# Autodesk Inventor assembly: upper_body
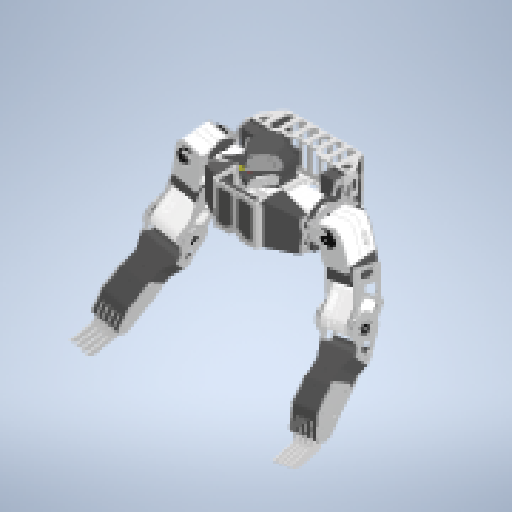
[picture p0: Inventor's stored thumbnail of the model, 512x512]
Saved by Autodesk Inventor 2024.1 (Build 281209000, 209)
## iProperties
Created: 2024-02-14
Part Number: upper_body
Document SubType Name: Assembly
Designer: hibik
Author: hibik
## Documents named in this file (3)
- C:\Users\hibik\Desktop\ロボメカ\HR\2024.02.11 Rl\02.11 ProtType\upper_body.iam
- C:\Users\hibik\Desktop\ロボメカ\HR\2024.02.11 Rl\02.11 ProtType\chest.iam
- C:\Users\hibik\Desktop\ロボメカ\HR\2024.02.11 Rl\02.11 ProtType\arm.iam
## Components (3 placed, 2 different names)
1. chest:1 [sub-assembly] — 挿入:1, 挿入:2
2. arm:1 [sub-assembly] — 挿入:1
3. arm:2 [sub-assembly] — 挿入:2
## Relationships (2: Insert 2)
- 挿入:1 [Insert]: chest:1 ↔ arm:1
- 挿入:2 [Insert]: chest:1 ↔ arm:2
